# Autodesk Inventor assembly: Dumber_2022
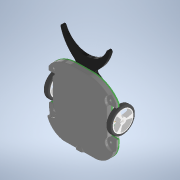
[picture p0: Inventor's stored thumbnail of the model, 180x180]
Saved by Autodesk Inventor 2021 (Build 250183000, 183)
## iProperties
Created: 2022-05-24
Part Number: Dumber_2022
Document SubType Name: Assembly
Designer: dimercur
Author: dimercur
## Documents named in this file (6)
- \\tsclient\dimercur\Travail\git\dumber\hardware\meca\Dumber_2022\Dumber_2022.iam
- \\tsclient\dimercur\Travail\git\dumber\hardware\meca\Dumber_2022\Pieces\coque_inf.ipt
- \\tsclient\dimercur\Travail\git\dumber\hardware\meca\Dumber_2022\Pieces\dumber-v3.iam
- \\tsclient\dimercur\Travail\git\dumber\hardware\meca\Dumber_2022\Pieces\coque_sup_v2-2.ipt
- \\tsclient\dimercur\Travail\git\dumber\hardware\meca\Dumber_2022\Pieces\PCB_ecran_Kicad_Final.iam
- \\tsclient\dimercur\Travail\git\dumber\hardware\meca\Dumber_2022\Pieces\Pince.ipt
## Components (5 placed, 5 different names)
1. coque_inf:1 — Placage:2, Placage:3, Placage:4, Placage:6, Placage:7
2. dumber-v3:1 [sub-assembly] — Placage:1, Angle:1, Affleurement:1, Placage:2, Placage:3, Placage:4, Placage:5, Placage:11, Placage:12, Placage:13
3. coque_sup_v2-2:1 — Placage:5, Placage:6, Placage:7, Placage:8, Placage:9, Placage:10
4. PCB_ecran_Kicad_Final:1 [sub-assembly] — Placage:8, Placage:9, Placage:10
5. Pince:1 — Placage:11, Placage:12, Placage:13
## Relationships (15: Mate 13, Angle 1, Flush 1)
- Placage:1 [Mate]: dumber-v3:1
- Angle:1 (0 deg): dumber-v3:1
- Affleurement:1 [Flush]: dumber-v3:1
- Placage:2 [Mate]: coque_inf:1 ↔ dumber-v3:1
- Placage:3 [Mate]: coque_inf:1 ↔ dumber-v3:1
- Placage:4 [Mate]: coque_inf:1 ↔ dumber-v3:1
- Placage:5 [Mate]: dumber-v3:1 ↔ coque_sup_v2-2:1
- Placage:6 [Mate]: coque_inf:1 ↔ coque_sup_v2-2:1
- Placage:7 [Mate]: coque_inf:1 ↔ coque_sup_v2-2:1
- Placage:8 [Mate]: coque_sup_v2-2:1 ↔ PCB_ecran_Kicad_Final:1
- Placage:9 [Mate]: coque_sup_v2-2:1 ↔ PCB_ecran_Kicad_Final:1
- Placage:10 [Mate]: coque_sup_v2-2:1 ↔ PCB_ecran_Kicad_Final:1
- Placage:11 [Mate]: dumber-v3:1 ↔ Pince:1
- Placage:12 [Mate]: dumber-v3:1 ↔ Pince:1
- Placage:13 [Mate]: dumber-v3:1 ↔ Pince:1
